# Autodesk Inventor assembly: InternalBottomMoldAssembly
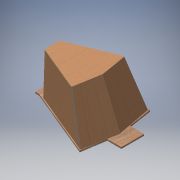
[picture p0: Inventor's stored thumbnail of the model, 180x180]
Saved by Autodesk Inventor 2019 (Build 230136000, 136)
## iProperties
Company: FABLAB Torino
Created: 2019-01-04
Part Number: InternalBottomMoldAssembly
Document SubType Name: Assembly
Designer: Giancarlo Bacchio
Project: La Panca - Flower Vase
Mass: 72304.3 g
Surface Area: 89186 cm^2
Volume: 48627 cm^3
Density: 1.48692 g/cm^3
Author: Giancarlo Bacchio
Title: La Panca - Flower Vase
Subject: Mold Structure
## Documents named in this file (6)
- D:\Giancarlo Bacchio\Documenti\00 - Progetti\30-Inventor\flower vase\InternalBottomMoldAssembly.iam
- D:\Giancarlo Bacchio\Documenti\00 - Progetti\30-Inventor\flower vase\intenalFormerBottmAssembly.iam
- D:\Giancarlo Bacchio\Documenti\00 - Progetti\30-Inventor\flower vase\internalSupportBottom1.ipt
- D:\Giancarlo Bacchio\Documenti\00 - Progetti\30-Inventor\flower vase\internalSupportBottom2.ipt
- D:\Giancarlo Bacchio\Documenti\00 - Progetti\30-Inventor\flower vase\internalSupportBottom4.ipt
- D:\Giancarlo Bacchio\Documenti\00 - Progetti\30-Inventor\flower vase\internalSupportBottom3.ipt
## Components (10 placed, 5 different names)
1. internalSupportBottom1:1
2. internalSupportBottom2:1 — Flush:26, Flush:27, Flush:28, Flush:29, Flush:30, Flush:31, Flush:32, Flush:33, Mate:54, Mate:55, Mate:56, Flush:34, Mate:57, Mate:58, Flush:36, Flush:37, Flush:38, Mate:59
3. internalSupportBottom4:1 — Flush:28, Flush:29
4. internalSupportBottom4:2 — Flush:31, Mate:56, Flush:34
5. internalSupportBottom4:3 — Flush:32, Mate:57
6. internalSupportBottom4:4 — Flush:30, Mate:54, Mate:55
7. internalSupportBottom4:5 — Flush:33, Mate:58
8. internalSupportBottom3:1 — Flush:36, Flush:37
9. internalSupportBottom3:2 — Flush:38, Mate:59
10. intenalFormerBottmAssembly:1 [sub-assembly] — Flush:26, Flush:27
## Relationships (18: Flush 12, Mate 6)
- Flush:26: internalSupportBottom2:1 ↔ intenalFormerBottmAssembly:1
- Flush:27: internalSupportBottom2:1 ↔ intenalFormerBottmAssembly:1
- Flush:28: internalSupportBottom2:1 ↔ internalSupportBottom4:1
- Flush:29: internalSupportBottom2:1 ↔ internalSupportBottom4:1
- Flush:30: internalSupportBottom2:1 ↔ internalSupportBottom4:4
- Flush:31: internalSupportBottom2:1 ↔ internalSupportBottom4:2
- Flush:32: internalSupportBottom2:1 ↔ internalSupportBottom4:3
- Flush:33: internalSupportBottom2:1 ↔ internalSupportBottom4:5
- Mate:54: internalSupportBottom2:1 ↔ internalSupportBottom4:4
- Mate:55: internalSupportBottom2:1 ↔ internalSupportBottom4:4
- Mate:56: internalSupportBottom2:1 ↔ internalSupportBottom4:2
- Flush:34: internalSupportBottom2:1 ↔ internalSupportBottom4:2
- Mate:57: internalSupportBottom2:1 ↔ internalSupportBottom4:3
- Mate:58: internalSupportBottom2:1 ↔ internalSupportBottom4:5
- Flush:36: internalSupportBottom2:1 ↔ internalSupportBottom3:1
- Flush:37: internalSupportBottom2:1 ↔ internalSupportBottom3:1
- Flush:38: internalSupportBottom2:1 ↔ internalSupportBottom3:2
- Mate:59: internalSupportBottom2:1 ↔ internalSupportBottom3:2
